# Autodesk Inventor assembly: 1Servo_Module_HXT
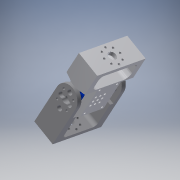
[picture p0: Inventor's stored thumbnail of the model, 180x180]
Saved by Autodesk Inventor 2018 (Build 220112000, 112)
## iProperties
Created: 2016-10-24
Part Number: 1Servo_Module_HXT
Document SubType Name: Assembly
Designer: Lucas
Author: Lucas
## Documents named in this file (11)
- D:\PhD\Teaching\Projects\CAD_Files\EDMO_Module_TGY_50090M\Assembly\EDMO_Module_TGY_50090M.iam
- D:\PhD\Teaching\Projects\CAD_Files\EDMO_Module_TGY_50090M\Workspace\DIN 125 - A 3,2.ipt
- D:\PhD\Teaching\Projects\CAD_Files\EDMO_Module_TGY_50090M\Workspace\DIN 985 - M3.ipt
- D:\PhD\Teaching\Projects\CAD_Files\EDMO_Module_TGY_50090M\Workspace\DIN 934 - M2 x 0,4.ipt
- D:\PhD\Teaching\Projects\CAD_Files\EDMO_Module_TGY_50090M\Workspace\DIN 912 - M2 x 0,4 x 20 x 19.ipt
- D:\PhD\Teaching\Projects\CAD_Files\EDMO_Module_TGY_50090M\Workspace\DIN 912 - M3 x 0,5 x 20 x 18,75.ipt
- D:\PhD\Teaching\Projects\CAD_Files\EDMO_Module_TGY_50090M\Workspace\Module_Arm.ipt
- D:\PhD\Teaching\Projects\CAD_Files\EDMO_Module_TGY_50090M\Workspace\Module_Cover.ipt
- D:\PhD\Teaching\Projects\CAD_Files\EDMO_Module_TGY_50090M\Workspace\Turnigy TGY-50090M Analog Servo.ipt
- D:\PhD\Teaching\Projects\CAD_Files\EDMO_Module_TGY_50090M\Workspace\Module_Body.ipt
- D:\PhD\Teaching\Projects\CAD_Files\EDMO_Module_TGY_50090M\Workspace\Servo_Horn_Cross_TGY.ipt
## Components (19 placed, 10 different names)
1. Module_Body:1 — Insert:4, Insert:5, Insert:49, Insert:50, Insert:55, Insert:56, Mate:5, Flush:1, Mate:6, Flush:2
2. DIN 125-1 A A 3,2:1 — Insert:4, Insert:106
3. DIN 125-1 A A 3,2:2 — Insert:5, Insert:7
4. DIN 985 - replaced by DIN EN ISO 10511 M3:1 — Insert:7, Insert:10
5. DIN 985 - replaced by DIN EN ISO 10511 M3:2 — Insert:10, Insert:48
6. DIN 125-1 A A 3,2:3 — Insert:48, Insert:107
7. DIN 125-1 A A 3,2:20 — Insert:34, Insert:108
8. DIN 985 - replaced by DIN EN ISO 10511 M3:3 — Insert:34
9. Module_Cover:1 — Insert:49, Insert:50, Insert:58, Insert:59, Insert:60, Insert:61
10. DIN 934 - replaced by DIN EN 24032/28673/28674 M2:2 — Insert:55
11. DIN 934 - replaced by DIN EN 24032/28673/28674 M2:1 — Insert:56
12. DIN 912 - replaced by DIN EN ISO 4762 M2 x 20:1 — Insert:58
13. DIN 912 - replaced by DIN EN ISO 4762 M2 x 20:2 — Insert:59
14. DIN 912 - replaced by DIN EN ISO 4762 M2 x 20:3 — Insert:60
15. DIN 912 - replaced by DIN EN ISO 4762 M2 x 20:4 — Insert:61
16. DIN 912 - replaced by DIN EN ISO 4762 M3 x 20:1 — Insert:106
17. Module_Arm:1 — Insert:107, Insert:108, Flush:2, Angle:1
18. Turnigy TGY-50090M Analog Servo:1 — Mate:5, Flush:1, Mate:6, Mate:7, Flush:3
19. Servo_Horn_Cross_TGY:1 — Mate:7, Flush:3, Angle:1
## Relationships (24: Insert 17, Mate 3, Flush 3, Angle 1)
- Insert:4: Module_Body:1 ↔ DIN 125-1 A A 3,2:1
- Insert:5: Module_Body:1 ↔ DIN 125-1 A A 3,2:2
- Insert:7: DIN 125-1 A A 3,2:2 ↔ DIN 985 - replaced by DIN EN ISO 10511 M3:1
- Insert:10: DIN 985 - replaced by DIN EN ISO 10511 M3:1 ↔ DIN 985 - replaced by DIN EN ISO 10511 M3:2
- Insert:34: DIN 125-1 A A 3,2:20 ↔ DIN 985 - replaced by DIN EN ISO 10511 M3:3
- Insert:48: DIN 985 - replaced by DIN EN ISO 10511 M3:2 ↔ DIN 125-1 A A 3,2:3
- Insert:49: Module_Body:1 ↔ Module_Cover:1
- Insert:50: Module_Body:1 ↔ Module_Cover:1
- Insert:55: Module_Body:1 ↔ DIN 934 - replaced by DIN EN 24032/28673/28674 M2:2
- Insert:56: Module_Body:1 ↔ DIN 934 - replaced by DIN EN 24032/28673/28674 M2:1
- Insert:58: Module_Cover:1 ↔ DIN 912 - replaced by DIN EN ISO 4762 M2 x 20:1
- Insert:59: Module_Cover:1 ↔ DIN 912 - replaced by DIN EN ISO 4762 M2 x 20:2
- Insert:60: Module_Cover:1 ↔ DIN 912 - replaced by DIN EN ISO 4762 M2 x 20:3
- Insert:61: Module_Cover:1 ↔ DIN 912 - replaced by DIN EN ISO 4762 M2 x 20:4
- Insert:106: DIN 125-1 A A 3,2:1 ↔ DIN 912 - replaced by DIN EN ISO 4762 M3 x 20:1
- Insert:107: DIN 125-1 A A 3,2:3 ↔ Module_Arm:1
- Insert:108: DIN 125-1 A A 3,2:20 ↔ Module_Arm:1
- Mate:5: Module_Body:1 ↔ Turnigy TGY-50090M Analog Servo:1
- Flush:1: Module_Body:1 ↔ Turnigy TGY-50090M Analog Servo:1
- Mate:6: Module_Body:1 ↔ Turnigy TGY-50090M Analog Servo:1
- Flush:2: Module_Body:1 ↔ Module_Arm:1
- Mate:7: Turnigy TGY-50090M Analog Servo:1 ↔ Servo_Horn_Cross_TGY:1
- Flush:3 (-5 mm): Turnigy TGY-50090M Analog Servo:1 ↔ Servo_Horn_Cross_TGY:1
- Angle:1 (-90 deg): Module_Arm:1 ↔ Servo_Horn_Cross_TGY:1
